# Autodesk Inventor assembly: solar_harvester_v2
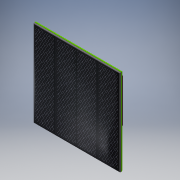
[picture p0: Inventor's stored thumbnail of the model, 180x180]
Saved by Autodesk Inventor 2018 (Build 220112000, 112)
## iProperties
Created: 2019-07-24
Part Number: solar_harvester_v2
Document SubType Name: Assembly
Designer: ZEUSLAP
Author: ZEUSLAP
## Documents named in this file (14)
- C:\data\solar-harvester\solar_harvester_165x165_MCP73871_BLM.iam
- C:\data\solar-harvester\parts\sp16_waterproof_connector\sp16-2P_female_back_nut_type.iam
- C:\data\solar-harvester\parts\sp16_waterproof_connector\parts\nut.ipt
- C:\data\solar-harvester\parts\sp16_waterproof_connector\parts\rubber_washer.ipt
- C:\data\solar-harvester\parts\18650_battery.ipt
- C:\data\solar-harvester\enclosure\front\solar_panel_frame.ipt
- C:\data\solar-harvester\parts\panels\solar_panel_165x165mm.ipt
- C:\data\solar-harvester\enclosure\back\back_lid_MCP73871_BLM.ipt
- C:\data\solar-harvester\parts\chargers\MCP73871_breakout_board_Shrinkwrap.ipt
- C:\data\solar-harvester\parts\battery_holders\Blossom BLM\BLOSSOM-BLM-18650-1PCS.iam
- C:\data\solar-harvester\enclosure\back\charger_holder_MCP73871.ipt
- C:\Users\ZEUSLAP\Documents\Inventor\Content Center Files\R2018\en-US\ISO 7049 - C-Z(2)\ISO 7049 - ST 2.9 x 6.5 - C - Z.ipt
- C:\Users\ZEUSLAP\Documents\Inventor\Content Center Files\R2018\en-US\SFS EN ISO 7045 Z\EN ISO 7045 - M3 x 8 - 4.8 - Z(3).ipt
- C:\Users\ZEUSLAP\Documents\Inventor\Content Center Files\R2018\en-US\ISO 4035(2)\ISO 4035 - M3 - ISO.ipt
## Components (60 placed, 13 different names)
1. solar_panel_165x165mm:1 — Mate:56, Mate:67, Mate:68
2. solar_panel_frame_136x110:1 — Mate:36, Mate:37, Mate:38, Angle:1, Mate:50, Mate:51, Mate:52, Mate:53, Angle:5, Mate:54, Mate:55, Mate:56, Mate:67, Mate:68, Mate:124, Mate:126, Mate:128, Mate:130, Mate:132, Mate:134, Mate:136, Mate:138, Mate:140, Mate:142, Mate:144, Mate:146, Mate:148, Mate:150, Mate:152, Mate:154, Mate:156, Mate:158, Mate:160, Mate:162, Mate:164, Mate:166, Mate:168
3. SP16-2P, female, back nut type:1 [sub-assembly] — Mate:31, Mate:32, Mate:34, Mate:37
4. nut:1 — Mate:32, Mate:38, Angle:1
5. rubber_washer:1 — Mate:31, Mate:34, Mate:36
6. back_lid_MCP73871_BLM:1 — Mate:50, Mate:51, Mate:52, Mate:53, Mate:57, Mate:58, Angle:6, Mate:62, Mate:65, Mate:66, Mate:69, Mate:71, Mate:73, Mate:75, Mate:77, Mate:78, Mate:79, Mate:80, Mate:81, Mate:82, Mate:83, Mate:84, Mate:85, Mate:86, Mate:87, Mate:88, Mate:89, Mate:90, Mate:91, Mate:92, Mate:93, Mate:94, Mate:95, Mate:96, Mate:97, Mate:98, Mate:99, Mate:100, Mate:101, Mate:102, Mate:103, Mate:104, Mate:105, Mate:106, Mate:107, Mate:108, Mate:109, Mate:110, Mate:111, Mate:112, Mate:113, Mate:114, Mate:115, Mate:116, Mate:117, Mate:118, Mate:119, Mate:120, Mate:121, Mate:122
7. 18650_battery:1 — Mate:59, Mate:60, Mate:61
8. MCP73871_breakout_board_Shrinkwrap:1 — Mate:62, Mate:63, Angle:7, Mate:64
9. BLOSSOM-BLM-18650-1PCS:1 [sub-assembly] — Mate:57, Mate:58, Angle:6, Mate:59, Mate:60, Mate:61, Mate:70, Mate:72
10. charger_holder_MCP73871:1 — Mate:63, Angle:7, Mate:64, Mate:65, Mate:66, Mate:74, Mate:76
11. ISO 7049 - C-Z ST 2.9 x 6.5 - C - Z:1 — Mate:69, Mate:70
12. ISO 7049 - C-Z ST 2.9 x 6.5 - C - Z:2 — Mate:71, Mate:72
13. ISO 7049 - C-Z ST 2.9 x 6.5 - C - Z:3 — Mate:73, Mate:74
14. ISO 7049 - C-Z ST 2.9 x 6.5 - C - Z:4 — Mate:75, Mate:76
15. SFS EN ISO 7045 Z M3 x 8 - 4.8 - Z:1 — Mate:77, Mate:78, Mate:123
16. SFS EN ISO 7045 Z M3 x 8 - 4.8 - Z:2 — Mate:79, Mate:80, Mate:151
17. SFS EN ISO 7045 Z M3 x 8 - 4.8 - Z:3 — Mate:81, Mate:82, Mate:155
18. SFS EN ISO 7045 Z M3 x 8 - 4.8 - Z:4 — Mate:83, Mate:84, Mate:125
19. SFS EN ISO 7045 Z M3 x 8 - 4.8 - Z:5 — Mate:85, Mate:86, Mate:129
20. SFS EN ISO 7045 Z M3 x 8 - 4.8 - Z:6 — Mate:87, Mate:88, Mate:157
21. SFS EN ISO 7045 Z M3 x 8 - 4.8 - Z:7 — Mate:89, Mate:90, Mate:161
22. SFS EN ISO 7045 Z M3 x 8 - 4.8 - Z:8 — Mate:91, Mate:92, Mate:165
23. SFS EN ISO 7045 Z M3 x 8 - 4.8 - Z:9 — Mate:93, Mate:94, Mate:137
24. SFS EN ISO 7045 Z M3 x 8 - 4.8 - Z:10 — Mate:95, Mate:96, Mate:141
25. SFS EN ISO 7045 Z M3 x 8 - 4.8 - Z:11 — Mate:97, Mate:98, Mate:145
26. SFS EN ISO 7045 Z M3 x 8 - 4.8 - Z:12 — Mate:99, Mate:100, Mate:147
27. SFS EN ISO 7045 Z M3 x 8 - 4.8 - Z:13 — Mate:101, Mate:102, Mate:143
28. SFS EN ISO 7045 Z M3 x 8 - 4.8 - Z:14 — Mate:103, Mate:104, Mate:139
29. SFS EN ISO 7045 Z M3 x 8 - 4.8 - Z:15 — Mate:105, Mate:106, Mate:135
30. SFS EN ISO 7045 Z M3 x 8 - 4.8 - Z:16 — Mate:107, Mate:108, Mate:167
31. SFS EN ISO 7045 Z M3 x 8 - 4.8 - Z:17 — Mate:109, Mate:110, Mate:163
32. SFS EN ISO 7045 Z M3 x 8 - 4.8 - Z:18 — Mate:111, Mate:112, Mate:159
33. SFS EN ISO 7045 Z M3 x 8 - 4.8 - Z:19 — Mate:113, Mate:114, Mate:131
34. SFS EN ISO 7045 Z M3 x 8 - 4.8 - Z:20 — Mate:115, Mate:116, Mate:127
35. SFS EN ISO 7045 Z M3 x 8 - 4.8 - Z:21 — Mate:117, Mate:118, Mate:133
36. SFS EN ISO 7045 Z M3 x 8 - 4.8 - Z:22 — Mate:119, Mate:120, Mate:153
37. SFS EN ISO 7045 Z M3 x 8 - 4.8 - Z:23 — Mate:121, Mate:122, Mate:149
38. ISO 4035 M3:1 — Mate:123, Mate:124
39. ISO 4035 M3:2 — Mate:125, Mate:126
40. ISO 4035 M3:3 — Mate:127, Mate:128
41. ISO 4035 M3:4 — Mate:129, Mate:130
42. ISO 4035 M3:5 — Mate:131, Mate:132
43. ISO 4035 M3:6 — Mate:133, Mate:134
44. ISO 4035 M3:7 — Mate:135, Mate:136
45. ISO 4035 M3:8 — Mate:137, Mate:138
46. ISO 4035 M3:9 — Mate:139, Mate:140
47. ISO 4035 M3:10 — Mate:141, Mate:142
48. ISO 4035 M3:11 — Mate:143, Mate:144
49. ISO 4035 M3:12 — Mate:145, Mate:146
50. ISO 4035 M3:13 — Mate:147, Mate:148
51. ISO 4035 M3:14 — Mate:149, Mate:150
52. ISO 4035 M3:15 — Mate:151, Mate:152
53. ISO 4035 M3:16 — Mate:153, Mate:154
54. ISO 4035 M3:17 — Mate:155, Mate:156
55. ISO 4035 M3:18 — Mate:157, Mate:158
56. ISO 4035 M3:19 — Mate:159, Mate:160
57. ISO 4035 M3:20 — Mate:161, Mate:162
58. ISO 4035 M3:21 — Mate:163, Mate:164
59. ISO 4035 M3:22 — Mate:165, Mate:166
60. ISO 4035 M3:23 — Mate:167, Mate:168
## Relationships (129: Mate 125, Angle 4)
- Mate:31: SP16-2P, female, back nut type:1 ↔ rubber_washer:1
- Mate:32: SP16-2P, female, back nut type:1 ↔ nut:1
- Mate:34: SP16-2P, female, back nut type:1 ↔ rubber_washer:1
- Mate:36: solar_panel_frame_136x110:1 ↔ rubber_washer:1
- Mate:37: solar_panel_frame_136x110:1 ↔ SP16-2P, female, back nut type:1
- Mate:38: solar_panel_frame_136x110:1 ↔ nut:1
- Angle:1 (0 deg): solar_panel_frame_136x110:1 ↔ nut:1
- Mate:50: solar_panel_frame_136x110:1 ↔ back_lid_MCP73871_BLM:1
- Mate:51: solar_panel_frame_136x110:1 ↔ back_lid_MCP73871_BLM:1
- Mate:52: solar_panel_frame_136x110:1 ↔ back_lid_MCP73871_BLM:1
- Mate:53: solar_panel_frame_136x110:1 ↔ back_lid_MCP73871_BLM:1
- Angle:5 (90 deg): solar_panel_frame_136x110:1
- Mate:54: solar_panel_frame_136x110:1
- Mate:55: solar_panel_frame_136x110:1
- Mate:56: solar_panel_165x165mm:1 ↔ solar_panel_frame_136x110:1
- Mate:57: back_lid_MCP73871_BLM:1 ↔ BLOSSOM-BLM-18650-1PCS:1
- Mate:58: back_lid_MCP73871_BLM:1 ↔ BLOSSOM-BLM-18650-1PCS:1
- Angle:6 (0 deg): back_lid_MCP73871_BLM:1 ↔ BLOSSOM-BLM-18650-1PCS:1
- Mate:59 (10 mm): 18650_battery:1 ↔ BLOSSOM-BLM-18650-1PCS:1
- Mate:60 (10 mm): 18650_battery:1 ↔ BLOSSOM-BLM-18650-1PCS:1
- Mate:61 (5 mm): 18650_battery:1 ↔ BLOSSOM-BLM-18650-1PCS:1
- Mate:62: back_lid_MCP73871_BLM:1 ↔ MCP73871_breakout_board_Shrinkwrap:1
- Mate:63: MCP73871_breakout_board_Shrinkwrap:1 ↔ charger_holder_MCP73871:1
- Angle:7 (270 deg): MCP73871_breakout_board_Shrinkwrap:1 ↔ charger_holder_MCP73871:1
- Mate:64: MCP73871_breakout_board_Shrinkwrap:1 ↔ charger_holder_MCP73871:1
- Mate:65: back_lid_MCP73871_BLM:1 ↔ charger_holder_MCP73871:1
- Mate:66: back_lid_MCP73871_BLM:1 ↔ charger_holder_MCP73871:1
- Mate:67 (0.25 mm): solar_panel_165x165mm:1 ↔ solar_panel_frame_136x110:1
- Mate:68 (0.25 mm): solar_panel_165x165mm:1 ↔ solar_panel_frame_136x110:1
- Mate:69: back_lid_MCP73871_BLM:1 ↔ ISO 7049 - C-Z ST 2.9 x 6.5 - C - Z:1
- Mate:70: BLOSSOM-BLM-18650-1PCS:1 ↔ ISO 7049 - C-Z ST 2.9 x 6.5 - C - Z:1
- Mate:71: back_lid_MCP73871_BLM:1 ↔ ISO 7049 - C-Z ST 2.9 x 6.5 - C - Z:2
- Mate:72: BLOSSOM-BLM-18650-1PCS:1 ↔ ISO 7049 - C-Z ST 2.9 x 6.5 - C - Z:2
- Mate:73: back_lid_MCP73871_BLM:1 ↔ ISO 7049 - C-Z ST 2.9 x 6.5 - C - Z:3
- Mate:74: charger_holder_MCP73871:1 ↔ ISO 7049 - C-Z ST 2.9 x 6.5 - C - Z:3
- Mate:75: back_lid_MCP73871_BLM:1 ↔ ISO 7049 - C-Z ST 2.9 x 6.5 - C - Z:4
- Mate:76: charger_holder_MCP73871:1 ↔ ISO 7049 - C-Z ST 2.9 x 6.5 - C - Z:4
- Mate:77: back_lid_MCP73871_BLM:1 ↔ SFS EN ISO 7045 Z M3 x 8 - 4.8 - Z:1
- Mate:78: back_lid_MCP73871_BLM:1 ↔ SFS EN ISO 7045 Z M3 x 8 - 4.8 - Z:1
- Mate:79: back_lid_MCP73871_BLM:1 ↔ SFS EN ISO 7045 Z M3 x 8 - 4.8 - Z:2
- Mate:80: back_lid_MCP73871_BLM:1 ↔ SFS EN ISO 7045 Z M3 x 8 - 4.8 - Z:2
- Mate:81: back_lid_MCP73871_BLM:1 ↔ SFS EN ISO 7045 Z M3 x 8 - 4.8 - Z:3
- Mate:82: back_lid_MCP73871_BLM:1 ↔ SFS EN ISO 7045 Z M3 x 8 - 4.8 - Z:3
- Mate:83: back_lid_MCP73871_BLM:1 ↔ SFS EN ISO 7045 Z M3 x 8 - 4.8 - Z:4
- Mate:84: back_lid_MCP73871_BLM:1 ↔ SFS EN ISO 7045 Z M3 x 8 - 4.8 - Z:4
- Mate:85: back_lid_MCP73871_BLM:1 ↔ SFS EN ISO 7045 Z M3 x 8 - 4.8 - Z:5
- Mate:86: back_lid_MCP73871_BLM:1 ↔ SFS EN ISO 7045 Z M3 x 8 - 4.8 - Z:5
- Mate:87: back_lid_MCP73871_BLM:1 ↔ SFS EN ISO 7045 Z M3 x 8 - 4.8 - Z:6
- Mate:88: back_lid_MCP73871_BLM:1 ↔ SFS EN ISO 7045 Z M3 x 8 - 4.8 - Z:6
- Mate:89: back_lid_MCP73871_BLM:1 ↔ SFS EN ISO 7045 Z M3 x 8 - 4.8 - Z:7
- Mate:90: back_lid_MCP73871_BLM:1 ↔ SFS EN ISO 7045 Z M3 x 8 - 4.8 - Z:7
- Mate:91: back_lid_MCP73871_BLM:1 ↔ SFS EN ISO 7045 Z M3 x 8 - 4.8 - Z:8
- Mate:92: back_lid_MCP73871_BLM:1 ↔ SFS EN ISO 7045 Z M3 x 8 - 4.8 - Z:8
- Mate:93: back_lid_MCP73871_BLM:1 ↔ SFS EN ISO 7045 Z M3 x 8 - 4.8 - Z:9
- Mate:94: back_lid_MCP73871_BLM:1 ↔ SFS EN ISO 7045 Z M3 x 8 - 4.8 - Z:9
- Mate:95: back_lid_MCP73871_BLM:1 ↔ SFS EN ISO 7045 Z M3 x 8 - 4.8 - Z:10
- Mate:96: back_lid_MCP73871_BLM:1 ↔ SFS EN ISO 7045 Z M3 x 8 - 4.8 - Z:10
- Mate:97: back_lid_MCP73871_BLM:1 ↔ SFS EN ISO 7045 Z M3 x 8 - 4.8 - Z:11
- Mate:98: back_lid_MCP73871_BLM:1 ↔ SFS EN ISO 7045 Z M3 x 8 - 4.8 - Z:11
- Mate:99: back_lid_MCP73871_BLM:1 ↔ SFS EN ISO 7045 Z M3 x 8 - 4.8 - Z:12
- Mate:100: back_lid_MCP73871_BLM:1 ↔ SFS EN ISO 7045 Z M3 x 8 - 4.8 - Z:12
- Mate:101: back_lid_MCP73871_BLM:1 ↔ SFS EN ISO 7045 Z M3 x 8 - 4.8 - Z:13
- Mate:102: back_lid_MCP73871_BLM:1 ↔ SFS EN ISO 7045 Z M3 x 8 - 4.8 - Z:13
- Mate:103: back_lid_MCP73871_BLM:1 ↔ SFS EN ISO 7045 Z M3 x 8 - 4.8 - Z:14
- Mate:104: back_lid_MCP73871_BLM:1 ↔ SFS EN ISO 7045 Z M3 x 8 - 4.8 - Z:14
- Mate:105: back_lid_MCP73871_BLM:1 ↔ SFS EN ISO 7045 Z M3 x 8 - 4.8 - Z:15
- Mate:106: back_lid_MCP73871_BLM:1 ↔ SFS EN ISO 7045 Z M3 x 8 - 4.8 - Z:15
- Mate:107: back_lid_MCP73871_BLM:1 ↔ SFS EN ISO 7045 Z M3 x 8 - 4.8 - Z:16
- Mate:108: back_lid_MCP73871_BLM:1 ↔ SFS EN ISO 7045 Z M3 x 8 - 4.8 - Z:16
- Mate:109: back_lid_MCP73871_BLM:1 ↔ SFS EN ISO 7045 Z M3 x 8 - 4.8 - Z:17
- Mate:110: back_lid_MCP73871_BLM:1 ↔ SFS EN ISO 7045 Z M3 x 8 - 4.8 - Z:17
- Mate:111: back_lid_MCP73871_BLM:1 ↔ SFS EN ISO 7045 Z M3 x 8 - 4.8 - Z:18
- Mate:112: back_lid_MCP73871_BLM:1 ↔ SFS EN ISO 7045 Z M3 x 8 - 4.8 - Z:18
- Mate:113: back_lid_MCP73871_BLM:1 ↔ SFS EN ISO 7045 Z M3 x 8 - 4.8 - Z:19
- Mate:114: back_lid_MCP73871_BLM:1 ↔ SFS EN ISO 7045 Z M3 x 8 - 4.8 - Z:19
- Mate:115: back_lid_MCP73871_BLM:1 ↔ SFS EN ISO 7045 Z M3 x 8 - 4.8 - Z:20
- Mate:116: back_lid_MCP73871_BLM:1 ↔ SFS EN ISO 7045 Z M3 x 8 - 4.8 - Z:20
- Mate:117: back_lid_MCP73871_BLM:1 ↔ SFS EN ISO 7045 Z M3 x 8 - 4.8 - Z:21
- Mate:118: back_lid_MCP73871_BLM:1 ↔ SFS EN ISO 7045 Z M3 x 8 - 4.8 - Z:21
- Mate:119: back_lid_MCP73871_BLM:1 ↔ SFS EN ISO 7045 Z M3 x 8 - 4.8 - Z:22
- Mate:120: back_lid_MCP73871_BLM:1 ↔ SFS EN ISO 7045 Z M3 x 8 - 4.8 - Z:22
- Mate:121: back_lid_MCP73871_BLM:1 ↔ SFS EN ISO 7045 Z M3 x 8 - 4.8 - Z:23
- Mate:122: back_lid_MCP73871_BLM:1 ↔ SFS EN ISO 7045 Z M3 x 8 - 4.8 - Z:23
- Mate:123: SFS EN ISO 7045 Z M3 x 8 - 4.8 - Z:1 ↔ ISO 4035 M3:1
- Mate:124: solar_panel_frame_136x110:1 ↔ ISO 4035 M3:1
- Mate:125: SFS EN ISO 7045 Z M3 x 8 - 4.8 - Z:4 ↔ ISO 4035 M3:2
- Mate:126: solar_panel_frame_136x110:1 ↔ ISO 4035 M3:2
- Mate:127: SFS EN ISO 7045 Z M3 x 8 - 4.8 - Z:20 ↔ ISO 4035 M3:3
- Mate:128: solar_panel_frame_136x110:1 ↔ ISO 4035 M3:3
- Mate:129: SFS EN ISO 7045 Z M3 x 8 - 4.8 - Z:5 ↔ ISO 4035 M3:4
- Mate:130: solar_panel_frame_136x110:1 ↔ ISO 4035 M3:4
- Mate:131: SFS EN ISO 7045 Z M3 x 8 - 4.8 - Z:19 ↔ ISO 4035 M3:5
- Mate:132: solar_panel_frame_136x110:1 ↔ ISO 4035 M3:5
- Mate:133: SFS EN ISO 7045 Z M3 x 8 - 4.8 - Z:21 ↔ ISO 4035 M3:6
- Mate:134: solar_panel_frame_136x110:1 ↔ ISO 4035 M3:6
- Mate:135: SFS EN ISO 7045 Z M3 x 8 - 4.8 - Z:15 ↔ ISO 4035 M3:7
- Mate:136: solar_panel_frame_136x110:1 ↔ ISO 4035 M3:7
- Mate:137: SFS EN ISO 7045 Z M3 x 8 - 4.8 - Z:9 ↔ ISO 4035 M3:8
- Mate:138: solar_panel_frame_136x110:1 ↔ ISO 4035 M3:8
- Mate:139: SFS EN ISO 7045 Z M3 x 8 - 4.8 - Z:14 ↔ ISO 4035 M3:9
- Mate:140: solar_panel_frame_136x110:1 ↔ ISO 4035 M3:9
- Mate:141: SFS EN ISO 7045 Z M3 x 8 - 4.8 - Z:10 ↔ ISO 4035 M3:10
- Mate:142: solar_panel_frame_136x110:1 ↔ ISO 4035 M3:10
- Mate:143: SFS EN ISO 7045 Z M3 x 8 - 4.8 - Z:13 ↔ ISO 4035 M3:11
- Mate:144: solar_panel_frame_136x110:1 ↔ ISO 4035 M3:11
- Mate:145: SFS EN ISO 7045 Z M3 x 8 - 4.8 - Z:11 ↔ ISO 4035 M3:12
- Mate:146: solar_panel_frame_136x110:1 ↔ ISO 4035 M3:12
- Mate:147: SFS EN ISO 7045 Z M3 x 8 - 4.8 - Z:12 ↔ ISO 4035 M3:13
- Mate:148: solar_panel_frame_136x110:1 ↔ ISO 4035 M3:13
- Mate:149: SFS EN ISO 7045 Z M3 x 8 - 4.8 - Z:23 ↔ ISO 4035 M3:14
- Mate:150: solar_panel_frame_136x110:1 ↔ ISO 4035 M3:14
- Mate:151: SFS EN ISO 7045 Z M3 x 8 - 4.8 - Z:2 ↔ ISO 4035 M3:15
- Mate:152: solar_panel_frame_136x110:1 ↔ ISO 4035 M3:15
- Mate:153: SFS EN ISO 7045 Z M3 x 8 - 4.8 - Z:22 ↔ ISO 4035 M3:16
- Mate:154: solar_panel_frame_136x110:1 ↔ ISO 4035 M3:16
- Mate:155: SFS EN ISO 7045 Z M3 x 8 - 4.8 - Z:3 ↔ ISO 4035 M3:17
- Mate:156: solar_panel_frame_136x110:1 ↔ ISO 4035 M3:17
- Mate:157: SFS EN ISO 7045 Z M3 x 8 - 4.8 - Z:6 ↔ ISO 4035 M3:18
- Mate:158: solar_panel_frame_136x110:1 ↔ ISO 4035 M3:18
- Mate:159: SFS EN ISO 7045 Z M3 x 8 - 4.8 - Z:18 ↔ ISO 4035 M3:19
- Mate:160: solar_panel_frame_136x110:1 ↔ ISO 4035 M3:19
- Mate:161: SFS EN ISO 7045 Z M3 x 8 - 4.8 - Z:7 ↔ ISO 4035 M3:20
- Mate:162: solar_panel_frame_136x110:1 ↔ ISO 4035 M3:20
- Mate:163: SFS EN ISO 7045 Z M3 x 8 - 4.8 - Z:17 ↔ ISO 4035 M3:21
- Mate:164: solar_panel_frame_136x110:1 ↔ ISO 4035 M3:21
- Mate:165: SFS EN ISO 7045 Z M3 x 8 - 4.8 - Z:8 ↔ ISO 4035 M3:22
- Mate:166: solar_panel_frame_136x110:1 ↔ ISO 4035 M3:22
- Mate:167: SFS EN ISO 7045 Z M3 x 8 - 4.8 - Z:16 ↔ ISO 4035 M3:23
- Mate:168: solar_panel_frame_136x110:1 ↔ ISO 4035 M3:23
